# Autodesk Inventor assembly: SteelM-StarS_MIR
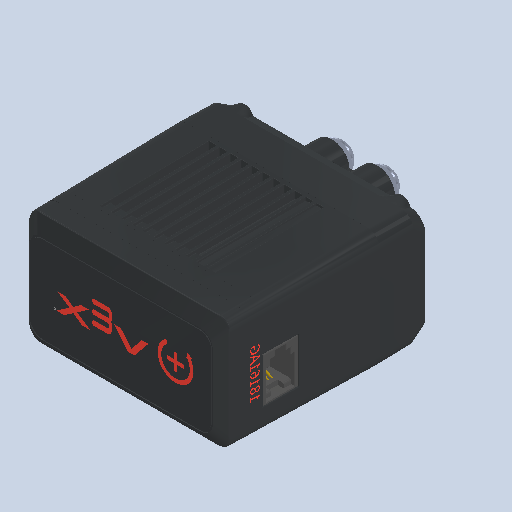
[picture p0: Inventor's stored thumbnail of the model, 512x512]
Saved by Autodesk Inventor 2023 (Build 270158000, 158)
## iProperties
Created: 2022-08-18
Part Number: SteelM-StarS_MIR
Document SubType Name: Assembly
Designer: Main Account
Author: ylu12
## Documents named in this file (4)
- D:\Documents\Inventor\VEX\Projects\SpinUpRobots\Flywheel\Mirror Dump\SteelM-StarS_MIR.iam
- D:\Documents\Inventor\VEX\Projects\SpinUpRobots\Flywheel\Mirror Dump\V5 Motor_MIR.ipt
- D:\Documents\Inventor\VEX\Library Backup\Library 1.4\Structure\Hardware\Screw Steel - Star\SScrew Star Smooth .500.ipt
- D:\Documents\Inventor\VEX\Library Backup\Library 1.4\Structure\Hardware\Screw Steel - Star.ipt
## Components (3 placed, 2 different names)
1. V5 Motor_MIR:1
2. SScrew Star Smooth .500:1
3. SScrew Star Smooth .500:2
## Named parameters: Thickness = 1.1938 mm
